# Autodesk Inventor assembly: box-iv stand connector
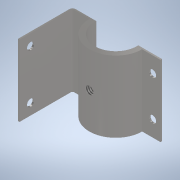
[picture p0: Inventor's stored thumbnail of the model, 180x180]
Saved by Autodesk Inventor 2020 (Build 240168000, 168)
## iProperties
Created: 2020-07-27
Part Number: box-iv stand connector
Document SubType Name: Assembly
Designer: Samuel
Author: Samuel
## Documents named in this file (4)
- C:\Users\Samuel\Desktop\box-iv stand connector.iam
- C:\Users\Samuel\Desktop\CNAF\CNAFgit\OpenHFNC\CAD\Prototype 3 (eng)\Plate B connector box-iv stand.ipt
- C:\Users\Samuel\Desktop\CNAF\CNAFgit\OpenHFNC\CAD\Prototype 3 (eng)\Plate A connector box-iv stand.ipt
- C:\Users\Samuel\Desktop\CNAF\CNAFgit\OpenHFNC\CAD\Prototype 3 (eng)\Half Pipe A53 - DN25-H45.ipt
## Components (3 placed, 3 different names)
1. Plate B connector box-iv stand:1 — Rigid:2
2. Plate A connector box-iv stand:1 — Rigid:1
3. Half Pipe A53 - DN25-H45:1 — Rigid:1, Rigid:2
## Relationships (2: WeldJoint 2)
- Rigid:1 [WeldJoint]: Plate A connector box-iv stand:1 ↔ Half Pipe A53 - DN25-H45:1
- Rigid:2 [WeldJoint]: Plate B connector box-iv stand:1 ↔ Half Pipe A53 - DN25-H45:1
